# Autodesk Inventor assembly: Main_Assembly
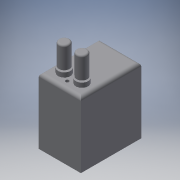
[picture p0: Inventor's stored thumbnail of the model, 180x180]
Saved by Autodesk Inventor 2017 (Build 210142000, 142)
## iProperties
Created: 2019-06-23
Part Number: Main_Assembly
Document SubType Name: Assembly
Designer: Mitch
Author: Mitch
## Documents named in this file (7)
- E:\Youtube Channel\Pojects\Fire Firework Controller\MECH\Main_Assembly.iam
- E:\Youtube Channel\Pojects\Fire Firework Controller\MECH\Battery_Box_Bottom.ipt
- E:\Youtube Channel\Pojects\Fire Firework Controller\MECH\Battery_Box_Top.ipt
- E:\Youtube Channel\Pojects\Fire Firework Controller\MECH\Terminal_Spacer.ipt
- E:\Youtube Channel\Pojects\Fire Firework Controller\MECH\Battery_Pack.ipt
- E:\Youtube Channel\Pojects\Fire Firework Controller\MECH\Terminal_Spacer_Top.ipt
- E:\Youtube Channel\Pojects\Fire Firework Controller\MECH\Battery Terminal.ipt
## Components (9 placed, 6 different names)
1. Battery_Box_Bottom:1 — Mate:5, Flush:1, Flush:2, Mate:6, Mate:7, Mate:8
2. Battery_Box_Top:1 — Mate:1, Mate:2, Mate:3, Mate:4, Mate:5, Flush:1, Flush:2, Mate:9, Mate:10, Mate:11, Mate:12
3. Terminal_Spacer:1 — Mate:1, Mate:3
4. Terminal_Spacer:2 — Mate:2, Mate:4
5. Battery_Pack:1 — Mate:6, Mate:7, Mate:8
6. Terminal_Spacer_Top:1 — Mate:10, Mate:12, Mate:13, Mate:15
7. Terminal_Spacer_Top:2 — Mate:9, Mate:11, Mate:14, Mate:16
8. Battery Terminal:1 — Mate:13, Mate:15
9. Battery Terminal:2 — Mate:14, Mate:16
## Relationships (18: Mate 16, Flush 2)
- Mate:1: Battery_Box_Top:1 ↔ Terminal_Spacer:1
- Mate:2: Battery_Box_Top:1 ↔ Terminal_Spacer:2
- Mate:3: Battery_Box_Top:1 ↔ Terminal_Spacer:1
- Mate:4: Battery_Box_Top:1 ↔ Terminal_Spacer:2
- Mate:5: Battery_Box_Bottom:1 ↔ Battery_Box_Top:1
- Flush:1: Battery_Box_Bottom:1 ↔ Battery_Box_Top:1
- Flush:2: Battery_Box_Bottom:1 ↔ Battery_Box_Top:1
- Mate:6: Battery_Box_Bottom:1 ↔ Battery_Pack:1
- Mate:7 (0.0508 mm): Battery_Box_Bottom:1 ↔ Battery_Pack:1
- Mate:8: Battery_Box_Bottom:1 ↔ Battery_Pack:1
- Mate:9: Battery_Box_Top:1 ↔ Terminal_Spacer_Top:2
- Mate:10: Battery_Box_Top:1 ↔ Terminal_Spacer_Top:1
- Mate:11: Battery_Box_Top:1 ↔ Terminal_Spacer_Top:2
- Mate:12: Battery_Box_Top:1 ↔ Terminal_Spacer_Top:1
- Mate:13 (2.4638 mm): Terminal_Spacer_Top:1 ↔ Battery Terminal:1
- Mate:14 (2.4638 mm): Terminal_Spacer_Top:2 ↔ Battery Terminal:2
- Mate:15: Terminal_Spacer_Top:1 ↔ Battery Terminal:1
- Mate:16: Terminal_Spacer_Top:2 ↔ Battery Terminal:2
